# Autodesk Inventor assembly: A2017_T5_10
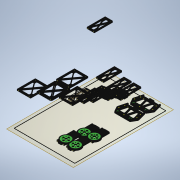
[picture p0: Inventor's stored thumbnail of the model, 180x180]
Saved by Autodesk Inventor 2022.3 (Build 263350000, 350)
## iProperties
Created: 2022-09-28
Part Number: A2017_T5_10
Document SubType Name: Assembly
Designer: Masato
Author: Masato
## Documents named in this file (7)
- C:\Users\Masato\Documents\Inventor\Inventor for CIT Brains\SUSTAINA-OP - cam\Cam\A2017_T5\A2017_T5_10.iam
- C:\Users\Masato\Documents\Inventor\Inventor for CIT Brains\SUSTAINA-OP - cam\Cam\DisposableBoard.ipt
- C:\Users\Masato\Documents\Inventor\Inventor for CIT Brains\SUSTAINA-OP - cam\LowerBody\Leg_joint\Leg_joint_yaw_frame.ipt
- C:\Users\Masato\Documents\Inventor\Inventor for CIT Brains\SUSTAINA-OP - cam\LowerBody\Link\BackLink_diagonal.ipt
- C:\Users\Masato\Documents\Inventor\Inventor for CIT Brains\SUSTAINA-OP - cam\LowerBody\Link\FrontLink_diagonal.ipt
- C:\Users\Masato\Documents\Inventor\Inventor for CIT Brains\SUSTAINA-OP - cam\UpperBody\UpperBody_horn_frame.ipt
- C:\Users\Masato\Documents\Inventor\Inventor for CIT Brains\SUSTAINA-OP - cam\UpperBody\Trunk\Trunk_lower_side_frame.ipt
## Components (22 placed, 6 different names)
1. DisposableBoard:1 — フラッシュ:1, フラッシュ:2, フラッシュ:3, フラッシュ:4
2. Leg_joint_yaw_frame:1
3. Leg_joint_yaw_frame:2
4. Leg_joint_yaw_frame:3
5. Leg_joint_yaw_frame:4
6. BackLink_diagonal:1
7. BackLink_diagonal:2
8. BackLink_diagonal:3
9. BackLink_diagonal:4
10. BackLink_diagonal:5
11. BackLink_diagonal:6
12. BackLink_diagonal:7
13. FrontLink_diagonal:1
14. FrontLink_diagonal:2
15. FrontLink_diagonal:3
16. FrontLink_diagonal:4
17. FrontLink_diagonal:5
18. UpperBody_horn_frame:1
19. UpperBody_horn_frame:2
20. UpperBody_horn_frame:3
21. Trunk_lower_side_frame:1
22. Trunk_lower_side_frame:2
## Relationships (4: Flush 4)
- フラッシュ:1 [Flush]: DisposableBoard:1
- フラッシュ:2 [Flush]: DisposableBoard:1
- フラッシュ:3 [Flush]: DisposableBoard:1
- フラッシュ:4 [Flush]: DisposableBoard:1
